# Autodesk Inventor assembly: Wheel Assembly
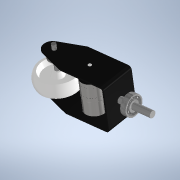
[picture p0: Inventor's stored thumbnail of the model, 180x180]
Saved by Autodesk Inventor 2020 (Build 240168000, 168)
## iProperties
Created: 2022-07-01
Part Number: Wheel Assembly
Document SubType Name: Assembly
Designer: karimi2
Author: karimi2
## Documents named in this file (8)
- C:\Users\karimi2\Documents\PROJECT\src\Wheel Assembly.iam
- C:\Users\karimi2\Documents\PROJECT\src\New frame.ipt
- C:\Users\karimi2\Documents\PROJECT\src\GearedDCmotor.ipt
- C:\Users\karimi2\Documents\PROJECT\src\wheelshaftGenerated.ipt
- C:\Users\karimi2\Documents\PROJECT\src\casterwheel.ipt
- C:\Users\karimi2\Documents\PROJECT\src\Wheel Assembly\Design Accelerator\Synchronous Belts Transmission1.iam
- C:\Users\karimi2\Documents\PROJECT\src\Bearing M8.iam
- C:\Users\karimi2\Documents\PROJECT\src\Shaft 8mm.ipt
## Components (7 placed, 7 different names)
1. New frame:1 — Mate:1, Mate:2, Mate:3, Mate:4, Mate:6, Mate:13, Rigid:3
2. GearedDCmotor:1 — Mate:1, Mate:2, Mate:11
3. Shaft:1 — Mate:3, Mate:4, Mate:5, Mate:12
4. casterwheel:1 — Mate:5, Mate:6
5. Synchronous Belts Transmission:2 [sub-assembly] — Mate:11, Mate:12, Mate:13
6. Shaft 8mm:1 — Rigid:3, Rotational:1
7. Bearing M8:1 [sub-assembly] — Rotational:1
## Relationships (11: Mate 9, WeldJoint 1, RevoluteJoint 1)
- Mate:1: New frame:1 ↔ GearedDCmotor:1
- Mate:2 (-40 mm): New frame:1 ↔ GearedDCmotor:1
- Mate:3: New frame:1 ↔ Shaft:1
- Mate:4 (-9 mm): New frame:1 ↔ Shaft:1
- Mate:5: Shaft:1 ↔ casterwheel:1
- Mate:6 (10 mm): New frame:1 ↔ casterwheel:1
- Mate:11: GearedDCmotor:1 ↔ Synchronous Belts Transmission:2
- Mate:12: Shaft:1 ↔ Synchronous Belts Transmission:2
- Mate:13 (0.5 mm): New frame:1 ↔ Synchronous Belts Transmission:2
- Rigid:3 [WeldJoint]: New frame:1 ↔ Shaft 8mm:1
- Rotational:1 [RevoluteJoint] (-23 mm): Shaft 8mm:1 ↔ Bearing M8:1
